# Autodesk Inventor assembly: sprint 1
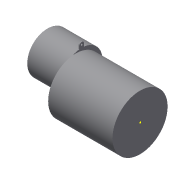
[picture p0: Inventor's stored thumbnail of the model, 180x180]
Saved by Autodesk Inventor 2019 (Build 230136000, 136)
## iProperties
Created: 2019-12-10
Part Number: sprint 1
Document SubType Name: Assembly
Designer: Sushma
Author: Sushma
## Documents named in this file (3)
- C:\Users\Sushma\Desktop\sprint 1.iam
- C:\Users\Sushma\Documents\roler.ipt
- C:\Users\Sushma\Documents\servo_motor.ipt
## Components (2 placed, 2 different names)
1. roler:1 — Mate:1
2. servo_motor:1 — Mate:1
## Relationships (1: Mate 1)
- Mate:1: roler:1 ↔ servo_motor:1
